# Autodesk Inventor assembly: Cube 1x1 V5
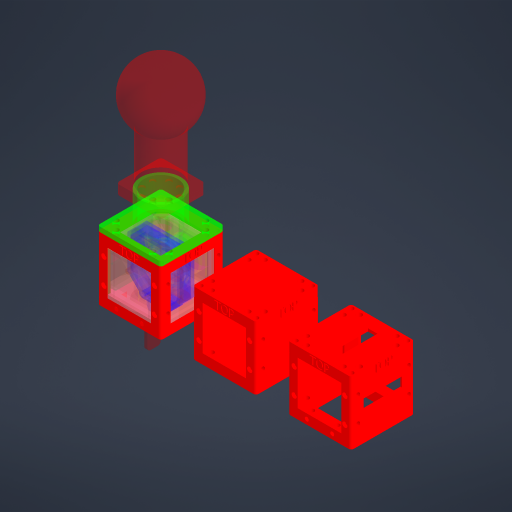
[picture p0: Inventor's stored thumbnail of the model, 512x512]
Saved by Autodesk Inventor 2023.4 (Build 274418000, 418)
## iProperties
Created: 2022-07-25
Part Number: Cube 1x1 V5
Document SubType Name: Assembly
Designer: xSibe
Author: xSibe
## Documents named in this file (54)
- C:\.Laptop\.Work\Projects\Project Protocube\Protocube\CAD, STL, OBJ Files\1 CAD\Cube 1x1 V5.iam
- C:\.Laptop\.Work\Projects\Project Protocube\Protocube\CAD, STL, OBJ Files\1 CAD\Cubes\Cube 1x1 Bottom V5.ipt
- C:\.Laptop\.Work\Projects\Project Protocube\Protocube\CAD, STL, OBJ Files\1 CAD\Cubes\Cube 1x1 Top V5.ipt
- C:\.Laptop\.Work\Projects\Project Protocube\Protocube\CAD, STL, OBJ Files\1 CAD\Lense\One Inch Lense Holder (V5).ipt
- C:\.Laptop\.Work\Projects\Project Protocube\Protocube\CAD, STL, OBJ Files\1 CAD\Lense\Half Inch Lense Holder (V5).ipt
- C:\.Laptop\.Work\Projects\Project Protocube\Protocube\CAD, STL, OBJ Files\1 CAD\Objective\Objective Mount.ipt
- C:\.Laptop\.Work\Projects\Project Protocube\Protocube\CAD, STL, OBJ Files\1 CAD\Mirror\Mirror Base Vertical.ipt
- C:\.Laptop\.Work\Projects\Project Protocube\Protocube\CAD, STL, OBJ Files\1 CAD\Mirror\Mirror Plate Vertical.ipt
- C:\.Laptop\.Work\Projects\Project Protocube\Protocube\CAD, STL, OBJ Files\1 CAD\Dichroic\Dichroic Mirror Mount.ipt
- C:\.Laptop\.Work\Projects\Project Protocube\Protocube\CAD, STL, OBJ Files\1 CAD\Attachments\Top Mount (SM1).ipt
- C:\.Laptop\.Work\Projects\Project Protocube\Protocube\CAD, STL, OBJ Files\1 CAD\Attachments\Flashlight Mount V1.ipt
- C:\.Laptop\.Work\Projects\Project Protocube\Protocube\CAD, STL, OBJ Files\1 CAD\Camera\Camera Mount Side.ipt
- C:\.Laptop\.Work\Projects\Project Protocube\Protocube\CAD, STL, OBJ Files\1 CAD\Panels\Panel Top 1x1.ipt
- C:\.Laptop\.Work\Projects\Project Protocube\Protocube\CAD, STL, OBJ Files\1 CAD\Panels\Panel Side 1x1.ipt
- C:\.Laptop\.Work\Projects\Project Protocube\Protocube\CAD, STL, OBJ Files\1 CAD\Panels\Panel Height 1x2.ipt
- C:\.Laptop\.Work\Projects\Project Protocube\Protocube\CAD, STL, OBJ Files\1 CAD\Attachments\Tunnel Vertical.ipt
- C:\.Laptop\.Work\Projects\Project Protocube\Protocube\CAD, STL, OBJ Files\1 CAD\Attachments\Tunnel Horizontal.ipt
- C:\.Laptop\.Work\Projects\Project Protocube\Protocube\CAD, STL, OBJ Files\1 CAD\Panels\Panel Side 1x2.ipt
- C:\.Laptop\.Work\Projects\Project Protocube\Protocube\CAD, STL, OBJ Files\1 CAD\Panels\Panel Side 1x3.ipt
- C:\.Laptop\.Work\Projects\Project Protocube\Protocube\CAD, STL, OBJ Files\1 CAD\Panels\Panel Side 1x4.ipt
- C:\.Laptop\.Work\Projects\Project Protocube\Protocube\CAD, STL, OBJ Files\1 CAD\Panels\Panel Side 1x5.ipt
- C:\.Laptop\.Work\Projects\Project Protocube\Protocube\CAD, STL, OBJ Files\1 CAD\Panels\Panel Top 1x2.ipt
- C:\.Laptop\.Work\Projects\Project Protocube\Protocube\CAD, STL, OBJ Files\1 CAD\Panels\Panel Top 1x3.ipt
- C:\.Laptop\.Work\Projects\Project Protocube\Protocube\CAD, STL, OBJ Files\1 CAD\Panels\Panel Top 1x4.ipt
- C:\.Laptop\.Work\Projects\Project Protocube\Protocube\CAD, STL, OBJ Files\1 CAD\Panels\Panel Top 1x5.ipt
- C:\.Laptop\.Work\Projects\Project Protocube\Protocube\CAD, STL, OBJ Files\1 CAD\Lense\SM1 Lense Holder (V5).ipt
- C:\.Laptop\.Work\Projects\Project Protocube\Protocube\CAD, STL, OBJ Files\1 CAD\Mirror\Mirror Base Horizontal.ipt
- C:\.Laptop\.Work\Projects\Project Protocube\Protocube\CAD, STL, OBJ Files\1 CAD\Mirror\Mirror Plate Horizontal.ipt
- C:\.Laptop\.Work\Projects\Project Protocube\Protocube\CAD, STL, OBJ Files\1 CAD\Tools\Baseplate V5 Press.ipt
- C:\.Laptop\.Work\Projects\Project Protocube\Protocube\CAD, STL, OBJ Files\1 CAD\Attachments\Cover Top (Full).ipt
- C:\.Laptop\.Work\Projects\Project Protocube\Protocube\CAD, STL, OBJ Files\1 CAD\Tools\Laser Alignment Tool V1.ipt
- C:\.Laptop\.Work\Projects\Project Protocube\Protocube\CAD, STL, OBJ Files\1 CAD\Filter\Filter Mount (SM05).ipt
- C:\.Laptop\.Work\Projects\Project Protocube\Protocube\CAD, STL, OBJ Files\1 CAD\Filter\Filter Mount (SM1).ipt
- C:\.Laptop\.Work\Projects\Project Protocube\Protocube\CAD, STL, OBJ Files\1 CAD\Covers\Cover Side (Normal).ipt
- C:\.Laptop\.Work\Projects\Project Protocube\Protocube\CAD, STL, OBJ Files\1 CAD\Covers\Cover Top (Normal) Proto.ipt
- C:\.Laptop\.Work\Projects\Project Protocube\Protocube\CAD, STL, OBJ Files\1 CAD\Covers\Cover Side (Slotted).ipt
- C:\.Laptop\.Work\Projects\Project Protocube\Protocube\CAD, STL, OBJ Files\1 CAD\Covers\Cover Top (Slotted) Proto.ipt
- C:\.Laptop\.Work\Projects\Project Protocube\Protocube\CAD, STL, OBJ Files\1 CAD\Cubes\Cube 1x1 Top V5 Closed.ipt
- C:\.Laptop\.Work\Projects\Project Protocube\Protocube\CAD, STL, OBJ Files\1 CAD\Cubes\Cube 1x1 Bottom V5 Closed.ipt
- C:\.Laptop\.Work\Projects\Project Protocube\Protocube\CAD, STL, OBJ Files\1 CAD\Cubes\Cube 1x1 Bottom V5 Closed Slotted.ipt
- C:\.Laptop\.Work\Projects\Project Protocube\Protocube\CAD, STL, OBJ Files\1 CAD\Cubes\Cube 1x1 Top V5 Closed Slotted.ipt
- C:\.Laptop\.Work\Projects\Project Protocube\Protocube\CAD, STL, OBJ Files\1 CAD\Lense\Half Inch Lense Holder Cover (V5).ipt
- C:\.Laptop\.Work\Projects\Project Protocube\Protocube\CAD, STL, OBJ Files\1 CAD\Lense\One Inch Lense Holder Cover (V5).ipt
- C:\.Laptop\.Work\Projects\Project Protocube\Protocube\CAD, STL, OBJ Files\1 CAD\Tools\Laser Alignment Tool V2.ipt
- C:\.Laptop\.Work\Projects\Project Protocube\Protocube\CAD, STL, OBJ Files\1 CAD\Lense\SM05 Lense Holder (V5).ipt
- C:\.Laptop\.Work\Projects\Project Protocube\Protocube\CAD, STL, OBJ Files\1 CAD\Laser\Laser Switch.ipt
- C:\.Laptop\.Work\Projects\Project Protocube\Protocube\CAD, STL, OBJ Files\1 CAD\Laser\Laser Holder (USB Laser).ipt
- C:\.Laptop\.Work\Projects\Project Protocube\Protocube\CAD, STL, OBJ Files\1 CAD\XYZ Stage\Z Stage Body V5.ipt
- C:\.Laptop\.Work\Projects\Project Protocube\Protocube\CAD, STL, OBJ Files\1 CAD\Attachments\Top Mount (SM05).ipt
- C:\.Laptop\.Work\Projects\Project Protocube\Protocube\CAD, STL, OBJ Files\1 CAD\Tools\Cube 1x1 V5 Bot Press.ipt
- C:\.Laptop\.Work\Projects\Project Protocube\Protocube\CAD, STL, OBJ Files\1 CAD\Tools\Cube 1x1 V5 Top Press.ipt
- C:\.Laptop\.Work\Projects\Project Protocube\Protocube\CAD, STL, OBJ Files\1 CAD\Filter\Filter Adapter (SM1).ipt
- C:\.Laptop\.Work\Projects\Project Protocube\Protocube\CAD, STL, OBJ Files\1 CAD\Filter\Filter Adapter (SM05).ipt
- C:\.Laptop\.Work\Projects\Project Protocube\Protocube\CAD, STL, OBJ Files\1 CAD\Laser\Laser Holder (Smaller Laser).ipt
## Components (53 placed, 53 different names)
1. Cube 1x1 Top V5:1 — Mate:1, Mate:2, Mate:3, Mate:4, Mate:5, Mate:6, Mate:40, Flush:23, Flush:24, Mate:60, Mate:61, Mate:62, Mate:63, Mate:64, Mate:65
2. Cube 1x1 Bottom V5:1 — Mate:1, Mate:2, Mate:3, Mate:9, Mate:10, Mate:11, Mate:39, Flush:21
3. Cube 1x1 Top V5 Closed:1 — Mate:40, Flush:23, Flush:24, Mate:41, Mate:42, Mate:43
4. Cube 1x1 Bottom V5 Closed:1 — Mate:41, Mate:42, Mate:43, Mate:54, Mate:55, Mate:56
5. Cube 1x1 Top V5 Closed Slotted:1 — Mate:51, Mate:52, Mate:53
6. Cube 1x1 Bottom V5 Closed Slotted:1 — Mate:51, Mate:52, Mate:53, Mate:54, Mate:55, Mate:56
7. Z Stage Body V5:1
8. Laser Alignment Tool V1:1 — Flush:18
9. Laser Alignment Tool V2:1
10. Baseplate V5 Press:1 — Flush:15
11. Cube 1x1 V5 Bot Press:1
12. Cube 1x1 V5 Top Press:1
13. Laser Switch:1
14. Half Inch Lense Holder Cover (V5):1
15. One Inch Lense Holder Cover (V5):1
16. Half Inch Lense Holder (V5):1
17. One Inch Lense Holder (V5):1 — Flush:1
18. Laser Holder (USB Laser):1
19. Laser Holder (Smaller Laser):1
20. SM05 Lense Holder (V5):1
21. SM1 Lense Holder (V5):1
22. Filter Mount (SM05):1 — Flush:19
23. Filter Mount (SM1):1
24. Tunnel Vertical:1 — Flush:10
25. Tunnel Horizontal:1 — Flush:11
26. Mirror Base Vertical:1 — Flush:5
27. Mirror Plate Vertical:1
28. Mirror Base Horizontal:1 — Flush:12, Flush:14
29. Mirror Plate Horizontal:1 — Mate:38, Flush:13, Flush:14
30. Dichroic Mirror Mount:1 — Flush:6
31. Camera Mount Side:1 — Flush:7
32. Objective Mount:1 — Flush:4
33. Filter Adapter (SM1):1
34. Filter Adapter (SM05):1
35. Top Mount (SM1):1 — Mate:4, Mate:5, Mate:6
36. Top Mount (SM05):1 — Mate:60, Mate:61, Mate:62
37. Flashlight Mount V1:1 — Mate:63, Mate:64, Mate:65
38. Cover Top (Full):1 — Flush:17
39. Cover Side (Normal):1 — Flush:20, Mate:39, Flush:21
40. Cover Side (Slotted):1
41. Cover Top (Normal) Proto:1 — Flush:22
42. Cover Top (Slotted) Proto:1
43. Panel Height 1x2:1 — Mate:9, Mate:10, Mate:11
44. Panel Top 1x1:1 — Flush:8, Mate:30, Mate:31
45. Panel Top 1x2:1 — Mate:21, Mate:22, Mate:29
46. Panel Top 1x3:1 — Mate:21, Mate:22, Mate:23, Mate:24, Mate:28, Mate:30
47. Panel Top 1x4:1 — Mate:23, Mate:24, Mate:25, Mate:26, Mate:27, Mate:29, Mate:31
48. Panel Top 1x5:1 — Mate:25, Mate:26, Mate:27, Mate:28
49. Panel Side 1x1:1 — Flush:9, Mate:32, Mate:33
50. Panel Side 1x2:1 — Mate:12, Mate:13, Mate:20
51. Panel Side 1x3:1 — Mate:12, Mate:13, Mate:14, Mate:15, Mate:19
52. Panel Side 1x4:1 — Mate:14, Mate:15, Mate:16, Mate:17, Mate:18, Mate:20, Mate:32
53. Panel Side 1x5:1 — Mate:16, Mate:17, Mate:18, Mate:19, Mate:33
## Relationships (70: Mate 49, Flush 21)
- Mate:1: Cube 1x1 Top V5:1 ↔ Cube 1x1 Bottom V5:1
- Mate:2: Cube 1x1 Top V5:1 ↔ Cube 1x1 Bottom V5:1
- Mate:3: Cube 1x1 Top V5:1 ↔ Cube 1x1 Bottom V5:1
- Flush:1: One Inch Lense Holder (V5):1
- Flush:4: Objective Mount:1
- Flush:5: Mirror Base Vertical:1
- Flush:6: Dichroic Mirror Mount:1
- Mate:4: Cube 1x1 Top V5:1 ↔ Top Mount (SM1):1
- Mate:5: Cube 1x1 Top V5:1 ↔ Top Mount (SM1):1
- Mate:6: Cube 1x1 Top V5:1 ↔ Top Mount (SM1):1
- Flush:7: Camera Mount Side:1
- Flush:8: Panel Top 1x1:1
- Flush:9: Panel Side 1x1:1
- Mate:9: Cube 1x1 Bottom V5:1 ↔ Panel Height 1x2:1
- Mate:10: Cube 1x1 Bottom V5:1 ↔ Panel Height 1x2:1
- Mate:11: Cube 1x1 Bottom V5:1 ↔ Panel Height 1x2:1
- Flush:10: Tunnel Vertical:1
- Flush:11: Tunnel Horizontal:1
- Mate:12: Panel Side 1x2:1 ↔ Panel Side 1x3:1
- Mate:13: Panel Side 1x2:1 ↔ Panel Side 1x3:1
- Mate:14: Panel Side 1x3:1 ↔ Panel Side 1x4:1
- Mate:15: Panel Side 1x3:1 ↔ Panel Side 1x4:1
- Mate:16: Panel Side 1x4:1 ↔ Panel Side 1x5:1
- Mate:17: Panel Side 1x4:1 ↔ Panel Side 1x5:1
- Mate:18: Panel Side 1x4:1 ↔ Panel Side 1x5:1
- Mate:19: Panel Side 1x3:1 ↔ Panel Side 1x5:1
- Mate:20: Panel Side 1x2:1 ↔ Panel Side 1x4:1
- Mate:21: Panel Top 1x2:1 ↔ Panel Top 1x3:1
- Mate:22: Panel Top 1x2:1 ↔ Panel Top 1x3:1
- Mate:23: Panel Top 1x3:1 ↔ Panel Top 1x4:1
- Mate:24: Panel Top 1x3:1 ↔ Panel Top 1x4:1
- Mate:25: Panel Top 1x4:1 ↔ Panel Top 1x5:1
- Mate:26: Panel Top 1x4:1 ↔ Panel Top 1x5:1
- Mate:27: Panel Top 1x4:1 ↔ Panel Top 1x5:1
- Mate:28: Panel Top 1x3:1 ↔ Panel Top 1x5:1
- Mate:29: Panel Top 1x2:1 ↔ Panel Top 1x4:1
- Mate:30: Panel Top 1x1:1 ↔ Panel Top 1x3:1
- Mate:31: Panel Top 1x1:1 ↔ Panel Top 1x4:1
- Mate:32: Panel Side 1x1:1 ↔ Panel Side 1x4:1
- Mate:33: Panel Side 1x1:1 ↔ Panel Side 1x5:1
- Flush:12: Mirror Base Horizontal:1
- Mate:38: Mirror Plate Horizontal:1
- Flush:13: Mirror Plate Horizontal:1
- Flush:14: Mirror Base Horizontal:1 ↔ Mirror Plate Horizontal:1
- Flush:15: Baseplate V5 Press:1
- Flush:17: Cover Top (Full):1
- Flush:18: Laser Alignment Tool V1:1
- Flush:19: Filter Mount (SM05):1
- Flush:20: Cover Side (Normal):1
- Mate:39: Cube 1x1 Bottom V5:1 ↔ Cover Side (Normal):1
- Flush:21: Cube 1x1 Bottom V5:1 ↔ Cover Side (Normal):1
- Flush:22: Cover Top (Normal) Proto:1
- Mate:40 (25 mm): Cube 1x1 Top V5:1 ↔ Cube 1x1 Top V5 Closed:1
- Flush:23: Cube 1x1 Top V5:1 ↔ Cube 1x1 Top V5 Closed:1
- Flush:24: Cube 1x1 Top V5:1 ↔ Cube 1x1 Top V5 Closed:1
- Mate:41: Cube 1x1 Top V5 Closed:1 ↔ Cube 1x1 Bottom V5 Closed:1
- Mate:42: Cube 1x1 Top V5 Closed:1 ↔ Cube 1x1 Bottom V5 Closed:1
- Mate:43: Cube 1x1 Top V5 Closed:1 ↔ Cube 1x1 Bottom V5 Closed:1
- Mate:51: Cube 1x1 Top V5 Closed Slotted:1 ↔ Cube 1x1 Bottom V5 Closed Slotted:1
- Mate:52: Cube 1x1 Top V5 Closed Slotted:1 ↔ Cube 1x1 Bottom V5 Closed Slotted:1
- Mate:53: Cube 1x1 Top V5 Closed Slotted:1 ↔ Cube 1x1 Bottom V5 Closed Slotted:1
- Mate:54 (25 mm): Cube 1x1 Bottom V5 Closed:1 ↔ Cube 1x1 Bottom V5 Closed Slotted:1
- Mate:55: Cube 1x1 Bottom V5 Closed:1 ↔ Cube 1x1 Bottom V5 Closed Slotted:1
- Mate:56: Cube 1x1 Bottom V5 Closed:1 ↔ Cube 1x1 Bottom V5 Closed Slotted:1
- Mate:60: Cube 1x1 Top V5:1 ↔ Top Mount (SM05):1
- Mate:61: Cube 1x1 Top V5:1 ↔ Top Mount (SM05):1
- Mate:62: Cube 1x1 Top V5:1 ↔ Top Mount (SM05):1
- Mate:63: Cube 1x1 Top V5:1 ↔ Flashlight Mount V1:1
- Mate:64: Cube 1x1 Top V5:1 ↔ Flashlight Mount V1:1
- Mate:65: Cube 1x1 Top V5:1 ↔ Flashlight Mount V1:1
